# Autodesk Inventor assembly: рама
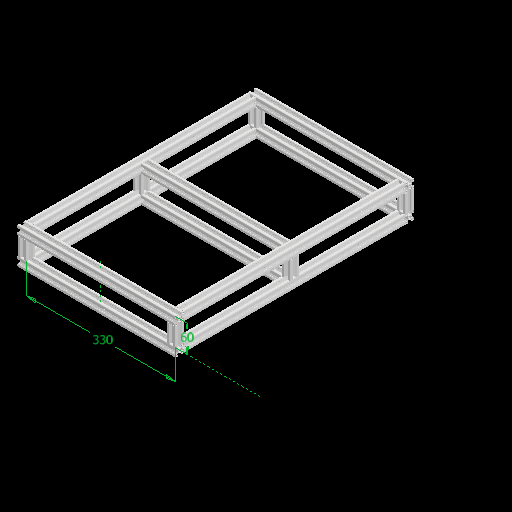
[picture p0: Inventor's stored thumbnail of the model, 512x512]
Saved by Autodesk Inventor 2025 (Build 290162000, 162)
## iProperties
Created: 2025-02-19
Part Number: рама
Document SubType Name: Assembly
Designer: volko
Mass: 1272.22 g
Surface Area: 8505.58 cm^2
Volume: 471.192 cm^3
Density: 2.7 g/cm^3
_SolveAssemblyDoc: Frame Generator Solve Assembly
_Version: 25.0.0
Author: volko
## Documents named in this file (3)
- C:\Users\volko\Desktop\диплом\Модели\детали\рама.iam
- C:\Users\volko\Desktop\диплом\Модели\детали\рама.ipt
- C:\Users\volko\Desktop\диплом\Модели\детали\рама\Frame\Frame 1740394805488.iam
## Components (2 placed, 2 different names)
1. рама:1 — Заподлицо:4, Заподлицо:6, Заподлицо:7
2. Frame 1740394805488:1 [sub-assembly] — Заподлицо:8, Заподлицо:9
## Relationships (5: Flush 5)
- Заподлицо:4 [Flush]: рама:1
- Заподлицо:6 [Flush] (-29 mm): рама:1
- Заподлицо:7 [Flush] (260 mm): рама:1
- Заподлицо:8 [Flush] (-39 mm): Frame 1740394805488:1
- Заподлицо:9 [Flush] (-290 mm): Frame 1740394805488:1
